# Autodesk Inventor assembly: Octanis1_Rover_Rev04_Musk
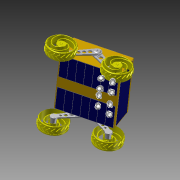
[picture p0: Inventor's stored thumbnail of the model, 180x180]
Saved by Autodesk Inventor 2014 SP1 (Build 180222100, 222)
## iProperties
Created: 2015-10-28
Part Number: Octanis1_Rover_Rev04_Musk
Document SubType Name: Assembly
Designer: Sam
Author: Sam
## Documents named in this file (32)
- C:\Users\Sam\Documents\GitHub\Octanis1-CAD\CAD_Rover_Rev04_Musk\Octanis1_Rover_Rev04_Musk.iam
- C:\Users\Sam\Documents\GitHub\Octanis1-CAD\CAD_Rover_Rev04_Musk\Imported Components\PTFE_Tube_ScrewClamp\PTFE_Tube_ScrewClamp.ipt
- C:\Users\Sam\Documents\GitHub\Octanis1-CAD\CAD_Rover_Rev04_Musk\Imported Components\PTFEStrutBushing\PTFEStrutBushing.ipt
- C:\Users\Sam\Documents\GitHub\Octanis1-CAD\CAD_Rover_Rev04_Musk\Imported Components\BasePlate\BasePlate.ipt
- C:\Users\Sam\Documents\GitHub\Octanis1-CAD\CAD_Rover_Rev04_Musk\Imported Components\InnerShaft\InnerShaft.ipt
- C:\Users\Sam\Documents\GitHub\Octanis1-CAD\CAD_Rover_Rev04_Musk\Imported Components\OuterShaft\OuterShaft.ipt
- C:\Users\Sam\Documents\GitHub\Octanis1-CAD\CAD_Rover_Rev04_Musk\Imported Components\ShaftGear_Inner_v2\ShaftGear_Inner_v2.ipt
- C:\Users\Sam\Documents\GitHub\Octanis1-CAD\CAD_Rover_Rev04_Musk\Imported Components\ShaftGear_Outer_Pinion_v2\ShaftGear_Outer_Pinion_v2.ipt
- C:\Users\Sam\Documents\GitHub\Octanis1-CAD\CAD_Rover_Rev04_Musk\Imported Components\ShaftGear_Outer_v2\ShaftGear_Outer_v2.ipt
- C:\Users\Sam\Documents\GitHub\Octanis1-CAD\CAD_Rover_Rev04_Musk\Imported Components\StrutGearbox\StrutGearbox.iam
- C:\Users\Sam\Documents\GitHub\Octanis1-CAD\CAD_Rover_Rev04_Musk\Imported Components\ShaftGear_Outer_v2\ShaftGear_Outer_v2_MIR.ipt
- C:\Users\Sam\Documents\Inventor\Content Center Files\R2014\en-US\Bearing 5 GOST 10058-90\Bearing 860024 GOST 10058-90.ipt
- C:\Users\Sam\Documents\GitHub\Octanis1-CAD\CAD_Rover_Rev04_Musk\Imported Components\StrutGearbox_Shaft\StrutGearbox_Shaft.ipt
- C:\Users\Sam\Documents\GitHub\Octanis1-CAD\CAD_Rover_Rev04_Musk\Imported Components\OuterStrut\OuterStrut.ipt
- C:\Users\Sam\Documents\GitHub\Octanis1-CAD\CAD_Rover_Rev04_Musk\Imported Components\OuterStrut\OuterStrut_MIR.ipt
- C:\Users\Sam\Documents\GitHub\Octanis1-CAD\CAD_Rover_Rev04_Musk\Imported Components\InnerStrut\InnerStrut.iam
- C:\Users\Sam\Documents\GitHub\Octanis1-CAD\CAD_Rover_Rev04_Musk\Imported Components\InnerStrut\InnerStrut_MIR.iam
- C:\Users\Sam\Documents\GitHub\Octanis1-CAD\CAD_Rover_Rev04_Musk\Imported Components\StrutMotorEnclosure\StrutMotorEnclosure.ipt
- C:\Users\Sam\Documents\GitHub\Octanis1-CAD\CAD_Rover_Rev04_Musk\Imported Components\WheelRight\WheelRight.iam
- C:\Users\Sam\Documents\GitHub\Octanis1-CAD\CAD_Rover_Rev04_Musk\Imported Components\WheelRight\WheelRight_MIR.iam
- C:\Users\Sam\Documents\GitHub\Octanis1-CAD\CAD_Rover_Rev04_Musk\Imported Components\WheelRight\WheelRight_MIR1.iam
- C:\Users\Sam\Documents\GitHub\Octanis1-CAD\CAD_Rover_Rev04_Musk\Imported Components\StrutMotorEnclosure\StrutMotorEnclosure_MIR.ipt
- C:\Users\Sam\Documents\GitHub\Octanis1-CAD\CAD_Rover_Rev04_Musk\Imported Components\InnerShaftClamp\InnerShaftClamp.ipt
- C:\Users\Sam\Documents\GitHub\Octanis1-CAD\CAD_Rover_Rev04_Musk\Imported Components\InnerShaftClamp\InnerShaftClamp_MIR1.ipt
- C:\Users\Sam\Documents\GitHub\Octanis1-CAD\CAD_Rover_Rev04_Musk\Imported Components\ShaftGear_Outer_Pinion_v2\ShaftGear_Outer_Pinion_v2_MIR4_MIR.ipt
- C:\Users\Sam\Documents\GitHub\Octanis1-CAD\CAD_Rover_Rev04_Musk\Imported Components\StrutGearbox\StrutGearbox_MIR4_MIR.iam
- C:\Users\Sam\Documents\GitHub\Octanis1-CAD\CAD_Rover_Rev04_Musk\Imported Components\StrutGearbox_Shaft\StrutGearbox_Shaft_MIR2_MIR.ipt
- C:\Users\Sam\Documents\GitHub\Octanis1-CAD\CAD_Rover_Rev04_Musk\Imported Components\FoamEnclosureBottom\FoamEnclosureBottom.ipt
- C:\Users\Sam\Documents\GitHub\Octanis1-CAD\CAD_Rover_Rev04_Musk\Imported Components\FoamEnclosureTop\FoamEnclosureTop.ipt
- C:\Users\Sam\Documents\GitHub\Octanis1-CAD\CAD_Rover_Rev04_Musk\Imported Components\TopInstrumentEnclosure\TopInstrumentEnclosure.ipt
- C:\Users\Sam\Documents\GitHub\Octanis1-CAD\CAD_Rover_Rev04_Musk\Imported Components\StereoscopicWebcamRig\StereoscopicWebcamRig_MIR_MIR.ipt
- C:\Users\Sam\Documents\GitHub\Octanis1-CAD\CAD_Rover_Rev04_Musk\Imported Components\SolarPanel\SolarPanel.iam
## Components (59 placed, 31 different names)
1. PTFE_Tube_ScrewClamp:1 — Rigid:4, Mate:2, Mate:3, Insert:3
2. PTFE_Tube_ScrewClamp:2 — Rigid:3, Insert:2
3. PTFE_Tube_ScrewClamp:3 — Rigid:3, Mate:16, Mate:17
4. PTFE_Tube_ScrewClamp:4 — Rigid:4
5. PTFEStrutBushing:1 — Insert:3, Insert:6, Tangent:1, Insert:18
6. BasePlate:1 — Mate:2, Mate:3, Mate:15, Mate:16, Mate:17, Mate:18, Angle:1, Tangent:1, Tangent:2, Mate:25, Mate:26, Angle:2, Angle:3, Mate:38, Mate:39, Angle:4, Angle:5, Angle:7
7. PTFEStrutBushing:2 — Insert:2, Insert:4, Tangent:2
8. InnerShaft:1 — Insert:5, Insert:9, Insert:15, Rotational:11
9. OuterShaft:1 — Insert:4, Insert:5, Insert:12, Insert:14
10. InnerShaft:2 — Insert:7, Insert:11, Insert:17, Rotational:12
11. OuterShaft:2 — Insert:6, Insert:7, Insert:13, Insert:16
12. ShaftGear_Inner_v2:1 — Insert:11
13. ShaftGear_Inner_v2:2 — Insert:9
14. ShaftGear_Outer_Pinion_v2:2 — Cylindrical:3, Mate:28
15. ShaftGear_Outer_v2:2 — Insert:12
16. StrutGearbox:1 [sub-assembly] — Mate:15, Rotational:1, Rotational:2, Angle:1, Mate:28, Angle:3
17. ShaftGear_Outer_v2_MIR:1 — Insert:13
18. Bearing 5 GOST 10058-90 860024:2 — Rotational:1, Cylindrical:2, Mate:31
19. Bearing 5 GOST 10058-90 860024:3 — Rotational:2, Cylindrical:1
20. StrutGearbox_Shaft:4 — Cylindrical:1, Cylindrical:2, Cylindrical:3, Mate:31
21. ShaftGear_Outer_Pinion_v2:3 — Mate:27
22. StrutGearbox:2 [sub-assembly] — Mate:18, Mate:27, Angle:2
23. Bearing 5 GOST 10058-90 860024:4 — Mate:30
24. Bearing 5 GOST 10058-90 860024:5
25. StrutGearbox_Shaft:5 — Mate:30
26. OuterStrut:1 — Insert:16, Cylindrical:13, Mate:22, Mate:23
27. OuterStrut_MIR:1 — Insert:14, Cylindrical:11, Mate:21
28. InnerStrut:1 [sub-assembly] — Insert:17, Cylindrical:14, Mate:24
29. InnerStrut_MIR:1 [sub-assembly] — Insert:15, Cylindrical:12, Mate:20
30. StrutMotorEnclosure:1 — Cylindrical:12, Mate:20, Rotational:8
31. StrutMotorEnclosure:2 — Cylindrical:11, Mate:21, Rotational:7
32. WheelRight:1 [sub-assembly] — Rotational:10
33. WheelRight:2 [sub-assembly] — Rotational:9
34. WheelRight_MIR:1 [sub-assembly] — Rotational:8
35. WheelRight_MIR1:1 [sub-assembly] — Rotational:7
36. StrutMotorEnclosure_MIR:1 — Cylindrical:14, Mate:24, Rotational:9
37. StrutMotorEnclosure_MIR:2 — Cylindrical:13, Mate:22, Mate:23, Rotational:10
38. InnerShaftClamp:1 — Rotational:12, Mate:25
39. InnerShaftClamp_MIR1:1 — Rotational:11, Mate:26
40. ShaftGear_Outer_Pinion_v2_MIR4_MIR:1 — Mate:34, Cylindrical:20
41. StrutGearbox_MIR4_MIR:1 [sub-assembly] — Mate:34, Rotational:15, Rotational:16, Mate:39, Angle:4
42. Bearing 5 GOST 10058-90 860024:8 — Mate:35, Rotational:15, Cylindrical:19
43. Bearing 5 GOST 10058-90 860024:9 — Rotational:16, Cylindrical:18
44. StrutGearbox_Shaft_MIR2_MIR:1 — Mate:35, Cylindrical:18, Cylindrical:19, Cylindrical:20
45. ShaftGear_Outer_Pinion_v2_MIR4_MIR:2
46. StrutGearbox_MIR4_MIR:2 [sub-assembly] — Mate:38, Angle:5
47. Bearing 5 GOST 10058-90 860024:10
48. Bearing 5 GOST 10058-90 860024:11
49. StrutGearbox_Shaft_MIR2_MIR:2
50. FoamEnclosureBottom:1 — Mate:43, Mate:44, Mate:56, Mate:58, Mate:59, Mate:60, Mate:61, Mate:62, Mate:63
51. FoamEnclosureTop:1 — Insert:18, Mate:40, Angle:6, Mate:41, Mate:42, Angle:7, Mate:43, Mate:44, Mate:45, Angle:8, Mate:46, Mate:47, Mate:48, Mate:50, Mate:51, Mate:52, Mate:53, Mate:54, Mate:55, Mate:57
52. TopInstrumentEnclosure:1 — Mate:40, Angle:6, Mate:41, Mate:42, Rigid:5
53. StereoscopicWebcamRig_MIR_MIR:1 — Rigid:5
54. SolarPanel:1 [sub-assembly] — Mate:45, Angle:8, Mate:46, Mate:47
55. SolarPanel:2 [sub-assembly] — Mate:48, Mate:50, Mate:51
56. SolarPanel:3 [sub-assembly] — Mate:52, Mate:53, Mate:54
57. SolarPanel:4 [sub-assembly] — Mate:55, Mate:56, Mate:57
58. SolarPanel:5 [sub-assembly] — Mate:58, Mate:59, Mate:60
59. SolarPanel:6 [sub-assembly] — Mate:61, Mate:62, Mate:63
## Relationships (104: Mate 46, CylindricalJoint 16, Insert 15, RevoluteJoint 14, Angle 8, WeldJoint 3, Tangent 2)
- Rigid:3 [WeldJoint] (4 mm): PTFE_Tube_ScrewClamp:2 ↔ PTFE_Tube_ScrewClamp:3
- Rigid:4 [WeldJoint] (4 mm): PTFE_Tube_ScrewClamp:1 ↔ PTFE_Tube_ScrewClamp:4
- Mate:2: PTFE_Tube_ScrewClamp:1 ↔ BasePlate:1
- Mate:3: PTFE_Tube_ScrewClamp:1 ↔ BasePlate:1
- Insert:2 (17 mm): PTFE_Tube_ScrewClamp:2 ↔ PTFEStrutBushing:2
- Insert:3 (-17 mm): PTFE_Tube_ScrewClamp:1 ↔ PTFEStrutBushing:1
- Insert:4 (15 mm): PTFEStrutBushing:2 ↔ OuterShaft:1
- Insert:5 (15 mm): InnerShaft:1 ↔ OuterShaft:1
- Insert:6 (-15 mm): PTFEStrutBushing:1 ↔ OuterShaft:2
- Insert:7 (-15 mm): InnerShaft:2 ↔ OuterShaft:2
- Insert:9 (9 mm): InnerShaft:1 ↔ ShaftGear_Inner_v2:2
- Insert:11 (9 mm): InnerShaft:2 ↔ ShaftGear_Inner_v2:1
- Mate:15: BasePlate:1 ↔ StrutGearbox:1
- Insert:12 (-42 mm): OuterShaft:1 ↔ ShaftGear_Outer_v2:2
- Insert:13: OuterShaft:2 ↔ ShaftGear_Outer_v2_MIR:1
- Rotational:1 [RevoluteJoint] (1 mm): StrutGearbox:1 ↔ Bearing 5 GOST 10058-90 860024:2
- Rotational:2 [RevoluteJoint] (-1 mm): StrutGearbox:1 ↔ Bearing 5 GOST 10058-90 860024:3
- Cylindrical:1: Bearing 5 GOST 10058-90 860024:3 ↔ StrutGearbox_Shaft:4
- Cylindrical:2: Bearing 5 GOST 10058-90 860024:2 ↔ StrutGearbox_Shaft:4
- Cylindrical:3: ShaftGear_Outer_Pinion_v2:2 ↔ StrutGearbox_Shaft:4
- [RevoluteJoint] (1 mm): StrutGearbox:2 ↔ Bearing 5 GOST 10058-90 860024:4
- [RevoluteJoint] (-1 mm): StrutGearbox:2 ↔ Bearing 5 GOST 10058-90 860024:5
- [CylindricalJoint]: Bearing 5 GOST 10058-90 860024:5 ↔ StrutGearbox_Shaft:5
- [CylindricalJoint]: Bearing 5 GOST 10058-90 860024:4 ↔ StrutGearbox_Shaft:5
- [CylindricalJoint]: ShaftGear_Outer_Pinion_v2:3 ↔ StrutGearbox_Shaft:5
- Insert:14: OuterShaft:1 ↔ OuterStrut_MIR:1
- Insert:15: InnerShaft:1 ↔ InnerStrut_MIR:1
- Insert:16: OuterShaft:2 ↔ OuterStrut:1
- Insert:17: InnerShaft:2 ↔ InnerStrut:1
- Mate:16: PTFE_Tube_ScrewClamp:3 ↔ BasePlate:1
- Mate:17: PTFE_Tube_ScrewClamp:3 ↔ BasePlate:1
- Mate:18: BasePlate:1 ↔ StrutGearbox:2
- Cylindrical:11: OuterStrut_MIR:1 ↔ StrutMotorEnclosure:2
- Cylindrical:12: InnerStrut_MIR:1 ↔ StrutMotorEnclosure:1
- Mate:20: InnerStrut_MIR:1 ↔ StrutMotorEnclosure:1
- Mate:21: OuterStrut_MIR:1 ↔ StrutMotorEnclosure:2
- Cylindrical:13: OuterStrut:1 ↔ StrutMotorEnclosure_MIR:2
- Cylindrical:14: InnerStrut:1 ↔ StrutMotorEnclosure_MIR:1
- Mate:22: OuterStrut:1 ↔ StrutMotorEnclosure_MIR:2
- Mate:23: OuterStrut:1 ↔ StrutMotorEnclosure_MIR:2
- Mate:24: InnerStrut:1 ↔ StrutMotorEnclosure_MIR:1
- Rotational:7 [RevoluteJoint] (-5 mm): StrutMotorEnclosure:2 ↔ WheelRight_MIR1:1
- Rotational:8 [RevoluteJoint] (5 mm): StrutMotorEnclosure:1 ↔ WheelRight_MIR:1
- Rotational:9 [RevoluteJoint] (5 mm): WheelRight:2 ↔ StrutMotorEnclosure_MIR:1
- Rotational:10 [RevoluteJoint] (5 mm): WheelRight:1 ↔ StrutMotorEnclosure_MIR:2
- Angle:1 (180 deg): BasePlate:1 ↔ StrutGearbox:1
- Tangent:1 (4 mm): PTFEStrutBushing:1 ↔ BasePlate:1
- Tangent:2 (4 mm): BasePlate:1 ↔ PTFEStrutBushing:2
- Rotational:11 [RevoluteJoint] (5 mm): InnerShaft:1 ↔ InnerShaftClamp_MIR1:1
- Rotational:12 [RevoluteJoint] (5 mm): InnerShaft:2 ↔ InnerShaftClamp:1
- Mate:25: BasePlate:1 ↔ InnerShaftClamp:1
- Mate:26: BasePlate:1 ↔ InnerShaftClamp_MIR1:1
- Mate:27 (2 mm): ShaftGear_Outer_Pinion_v2:3 ↔ StrutGearbox:2
- Mate:28 (2 mm): ShaftGear_Outer_Pinion_v2:2 ↔ StrutGearbox:1
- Mate:30 (3 mm): Bearing 5 GOST 10058-90 860024:4 ↔ StrutGearbox_Shaft:5
- Mate:31 (-3 mm): Bearing 5 GOST 10058-90 860024:2 ↔ StrutGearbox_Shaft:4
- Angle:2 (180 deg): BasePlate:1 ↔ StrutGearbox:2
- Angle:3 (180 deg): BasePlate:1 ↔ StrutGearbox:1
- Mate:34 (2 mm): ShaftGear_Outer_Pinion_v2_MIR4_MIR:1 ↔ StrutGearbox_MIR4_MIR:1
- Mate:35 (-3 mm): Bearing 5 GOST 10058-90 860024:8 ↔ StrutGearbox_Shaft_MIR2_MIR:1
- Rotational:15 [RevoluteJoint] (1 mm): StrutGearbox_MIR4_MIR:1 ↔ Bearing 5 GOST 10058-90 860024:8
- Rotational:16 [RevoluteJoint] (-1 mm): StrutGearbox_MIR4_MIR:1 ↔ Bearing 5 GOST 10058-90 860024:9
- Cylindrical:18: Bearing 5 GOST 10058-90 860024:9 ↔ StrutGearbox_Shaft_MIR2_MIR:1
- Cylindrical:19: Bearing 5 GOST 10058-90 860024:8 ↔ StrutGearbox_Shaft_MIR2_MIR:1
- Cylindrical:20: ShaftGear_Outer_Pinion_v2_MIR4_MIR:1 ↔ StrutGearbox_Shaft_MIR2_MIR:1
- [Mate] (2 mm): ShaftGear_Outer_Pinion_v2_MIR4_MIR:2 ↔ StrutGearbox_MIR4_MIR:2
- [Mate] (-3 mm): Bearing 5 GOST 10058-90 860024:10 ↔ StrutGearbox_Shaft_MIR2_MIR:2
- [RevoluteJoint] (1 mm): StrutGearbox_MIR4_MIR:2 ↔ Bearing 5 GOST 10058-90 860024:10
- [RevoluteJoint] (-1 mm): StrutGearbox_MIR4_MIR:2 ↔ Bearing 5 GOST 10058-90 860024:11
- [CylindricalJoint]: Bearing 5 GOST 10058-90 860024:11 ↔ StrutGearbox_Shaft_MIR2_MIR:2
- [CylindricalJoint]: Bearing 5 GOST 10058-90 860024:10 ↔ StrutGearbox_Shaft_MIR2_MIR:2
- [CylindricalJoint]: ShaftGear_Outer_Pinion_v2_MIR4_MIR:2 ↔ StrutGearbox_Shaft_MIR2_MIR:2
- Mate:38: BasePlate:1 ↔ StrutGearbox_MIR4_MIR:2
- Mate:39: BasePlate:1 ↔ StrutGearbox_MIR4_MIR:1
- Angle:4 (180 deg): BasePlate:1 ↔ StrutGearbox_MIR4_MIR:1
- Angle:5 (180 deg): BasePlate:1 ↔ StrutGearbox_MIR4_MIR:2
- Insert:18 (-5 mm): PTFEStrutBushing:1 ↔ FoamEnclosureTop:1
- Mate:40: FoamEnclosureTop:1 ↔ TopInstrumentEnclosure:1
- Angle:6 (0 deg): FoamEnclosureTop:1 ↔ TopInstrumentEnclosure:1
- Mate:41: FoamEnclosureTop:1 ↔ TopInstrumentEnclosure:1
- Mate:42: FoamEnclosureTop:1 ↔ TopInstrumentEnclosure:1
- Angle:7 (180 deg): BasePlate:1 ↔ FoamEnclosureTop:1
- Rigid:5 [WeldJoint]: TopInstrumentEnclosure:1 ↔ StereoscopicWebcamRig_MIR_MIR:1
- Mate:43: FoamEnclosureBottom:1 ↔ FoamEnclosureTop:1
- Mate:44: FoamEnclosureBottom:1 ↔ FoamEnclosureTop:1
- Mate:45: FoamEnclosureTop:1 ↔ SolarPanel:1
- Angle:8 (0 deg): FoamEnclosureTop:1 ↔ SolarPanel:1
- Mate:46 (15 mm): FoamEnclosureTop:1 ↔ SolarPanel:1
- Mate:47 (5 mm): FoamEnclosureTop:1 ↔ SolarPanel:1
- Mate:48 (5 mm): FoamEnclosureTop:1 ↔ SolarPanel:2
- Mate:50: FoamEnclosureTop:1 ↔ SolarPanel:2
- Mate:51: FoamEnclosureTop:1 ↔ SolarPanel:2
- Mate:52: FoamEnclosureTop:1 ↔ SolarPanel:3
- Mate:53 (5 mm): FoamEnclosureTop:1 ↔ SolarPanel:3
- Mate:54: FoamEnclosureTop:1 ↔ SolarPanel:3
- Mate:55: FoamEnclosureTop:1 ↔ SolarPanel:4
- Mate:56 (5 mm): FoamEnclosureBottom:1 ↔ SolarPanel:4
- Mate:57 (15 mm): FoamEnclosureTop:1 ↔ SolarPanel:4
- Mate:58: FoamEnclosureBottom:1 ↔ SolarPanel:5
- Mate:59: FoamEnclosureBottom:1 ↔ SolarPanel:5
- Mate:60 (5 mm): FoamEnclosureBottom:1 ↔ SolarPanel:5
- Mate:61: FoamEnclosureBottom:1 ↔ SolarPanel:6
- Mate:62: FoamEnclosureBottom:1 ↔ SolarPanel:6
- Mate:63 (5 mm): FoamEnclosureBottom:1 ↔ SolarPanel:6
## Named parameters: d117_d107 = 1 mm, d118_d108 = 132.155127 deg, d119_d109 = -1 mm, d120_d110 = -14.002081 deg, d121_d111 = 77.802605 deg, d122_d112 = 63.75021 mm, d123_d113 = -68.354603 deg, d124_d114 = 2.9805 mm, d125_d115 = 29.294959 deg, d126_d116 = 54.53464 mm, d232_d227 = 64.16971 mm, d233_d228 = -6.348946 deg, d234_d229 = 3.4 mm, d235_d230 = -5.598491 deg, d236_d231 = 54.11515 mm, d237_d220 = 2 mm, d238_d221 = -3 mm, d239_d222 = 1 mm, d240_d223 = 19.210094 deg, d241_d224 = -1 mm, d242_d225 = 91.319046 deg, d243_d226 = -78.457899 deg
